# Autodesk Inventor assembly: Assembly_XYZ_Stage_Micrometer_lightsheet
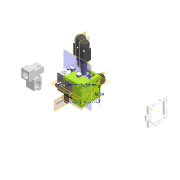
[picture p0: Inventor's stored thumbnail of the model, 180x180]
Saved by Autodesk Inventor 2022 (Build 260153000, 153)
## iProperties
Created: 2023-02-07
Part Number: Assembly_XYZ_Stage_Micrometer_lightsheet
Document SubType Name: Assembly
Designer: diederichbenedict
Author: diederichbenedict
## Documents named in this file (7)
- C:\Users\diederichbenedict\Dropbox\Dokumente\Promotion\PROJECTS\openUC2-CAD\INVENTOR\Assembly_XYZ_Stage_Micrometer_lightsheet.iam
- C:\Users\diederichbenedict\Dropbox\Dokumente\Promotion\PROJECTS\openUC2-CAD\INVENTOR\00_XYZstage_micro_LT-4047-S1.ipt
- C:\Users\diederichbenedict\Dropbox\Dokumente\Promotion\PROJECTS\openUC2-CAD\INVENTOR\00_Joy-IT-B20SHD4353_NEMA8_captive.ipt
- C:\Users\diederichbenedict\Dropbox\Dokumente\Promotion\PROJECTS\openUC2-CAD\INVENTOR\40_XYZstage_micrometer_motorized_nema8_cube.ipt
- C:\Users\diederichbenedict\Dropbox\Dokumente\Promotion\PROJECTS\openUC2-CAD\INVENTOR\40_XYZstage_micrometer_motorized_nema8_nanotec_adapter.ipt
- C:\Users\diederichbenedict\Dropbox\Dokumente\Promotion\PROJECTS\openUC2-CAD\INVENTOR\40_XYZstage_micrometer_motorized_nema8_nanotec_adapter_z.ipt
- C:\Users\diederichbenedict\Dropbox\Dokumente\Promotion\PROJECTS\openUC2-CAD\INVENTOR\10_Base_puzzle_v3.ipt
## Components (8 placed, 6 different names)
1. 00_XYZstage_micro_LT-4047-S1:1 — Passend:2, Passend:3, Winkel:1
2. 00_Joy-IT-B20SHD4353_NEMA8_captive:2
3. 00_Joy-IT-B20SHD4353_NEMA8_captive:1
4. 00_Joy-IT-B20SHD4353_NEMA8_captive:3
5. 40_XYZstage_micrometer_motorized_nema8_cube:1 — Passend:2, Passend:3, Winkel:1
6. 40_XYZstage_micrometer_motorized_nema8_nanotec_adapter:1
7. 40_XYZstage_micrometer_motorized_nema8_nanotec_adapter_z:1
8. 10_Base_puzzle_v3:1
## Relationships (6: Insert 3, Mate 2, Angle 1)
- [Insert]: 00_XYZstage_micro_LT-4047-S1:1 ↔ 00_Joy-IT-B20SHD4353_NEMA8_captive:1
- [Insert]: 00_XYZstage_micro_LT-4047-S1:1 ↔ 00_Joy-IT-B20SHD4353_NEMA8_captive:2
- [Insert]: 00_XYZstage_micro_LT-4047-S1:1 ↔ 00_Joy-IT-B20SHD4353_NEMA8_captive:3
- Passend:2 [Mate]: 00_XYZstage_micro_LT-4047-S1:1 ↔ 40_XYZstage_micrometer_motorized_nema8_cube:1
- Passend:3 [Mate]: 00_XYZstage_micro_LT-4047-S1:1 ↔ 40_XYZstage_micrometer_motorized_nema8_cube:1
- Winkel:1 [Angle] (90 deg): 00_XYZstage_micro_LT-4047-S1:1 ↔ 40_XYZstage_micrometer_motorized_nema8_cube:1
